# Autodesk Inventor assembly: Actual Robot
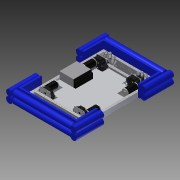
[picture p0: Inventor's stored thumbnail of the model, 180x180]
Saved by Autodesk Inventor 2014 SP1 (Build 180222100, 222)
## iProperties
Created: 2014-01-18
Part Number: Actual Robot
Document SubType Name: Assembly
Designer: Paul
Author: Paul
## Documents named in this file (3)
- C:\FRC_CAD\4859cad\Robot\Actual Robot\Actual Robot.iam
- C:\FRC_CAD\4859cad\Robot\KOP STEP\Electrical\Imported Components\ELEC_Battery_NP18-12B.iam\ELEC_Battery_NP18-12B.iam.iam
- ELEC_Battery_NP18-12B.iam
## Components (2 placed, 2 different names)
1. FrameAssembly :1 [sub-assembly] — Mate:1, Mate:2
2. ELEC_Battery_NP18-12B.iam:1 [sub-assembly] — Mate:1, Mate:2
## Relationships (2: Mate 2)
- Mate:1: FrameAssembly :1 ↔ ELEC_Battery_NP18-12B.iam:1
- Mate:2: FrameAssembly :1 ↔ ELEC_Battery_NP18-12B.iam:1
